# Autodesk Inventor assembly: каток сборка
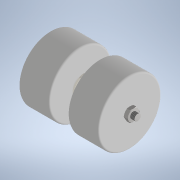
[picture p0: Inventor's stored thumbnail of the model, 180x180]
Saved by Autodesk Inventor 2020.1 (Build 241239000, 239)
## iProperties
Created: 2021-12-18
Part Number: каток сборка
Document SubType Name: Assembly
Designer: Ni3na
Author: Ni3na
## Documents named in this file (6)
- C:\Users\Ni3na\Documents\GitHub\TANK\3D-TANK\каток сборка.iam
- C:\Users\Ni3na\Documents\GitHub\TANK\3D-TANK\ось катка.ipt
- C:\Users\Ni3na\Documents\GitHub\TANK\3D-TANK\подшипник для катков.ipt
- C:\Users\Ni3na\Documents\GitHub\TANK\3D-TANK\каток.ipt
- C:\Users\Ni3na\Documents\Inventor\Content Center Files\R2020\ru-RU\AS 1112 (4)\AS 1112 - M4(2).ipt
- C:\Users\Ni3na\Documents\GitHub\TANK\3D-TANK\AS 1112 - M4(2).ipt
## Components (7 placed, 4 different names)
1. ось катка:1 — Жесткий:4
2. подшипник для катков:1 — Жесткий:1, Жесткий:3, Жесткий:4
3. подшипник для катков:2 — Жесткий:1, Жесткий:2
4. каток:1 — Жесткий:3, Жесткий:6
5. каток:2 — Жесткий:2, Жесткий:5
6. AS 1112 (4) - метрическая M4:3 — Жесткий:6
7. AS 1112 (4) - метрическая M4:2 — Жесткий:5
## Relationships (6: WeldJoint 6)
- Жесткий:1 [WeldJoint]: подшипник для катков:1 ↔ подшипник для катков:2
- Жесткий:2 [WeldJoint]: подшипник для катков:2 ↔ каток:2
- Жесткий:3 [WeldJoint]: подшипник для катков:1 ↔ каток:1
- Жесткий:4 [WeldJoint]: ось катка:1 ↔ подшипник для катков:1
- Жесткий:5 [WeldJoint]: каток:2 ↔ AS 1112 (4) - метрическая M4:2
- Жесткий:6 [WeldJoint]: каток:1 ↔ AS 1112 (4) - метрическая M4:3
